# Autodesk Inventor assembly: SPE3V1 Freno
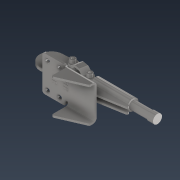
[picture p0: Inventor's stored thumbnail of the model, 180x180]
Saved by Autodesk Inventor 2021.2 (Build 252289000, 289)
## iProperties
Created: 2026-06-23
Part Number: SPE3V1 Freno
Document SubType Name: Assembly
Designer: nelso
Author: nelso
## Documents named in this file (9)
- C:\Users\Tecnica\OneDrive\Documentos\Mecanica\Soporte-Paciente-Espinografia\Workspace\SPE3V1 Freno.iam
- C:\Users\Tecnica\OneDrive\Documentos\Mecanica\Soporte-Paciente-Espinografia\Workspace\SP10V1 Estructura Freno.ipt
- C:\Users\Tecnica\OneDrive\Documentos\Mecanica\Soporte-Paciente-Espinografia\Workspace\SP9V1 Columna Freno.ipt
- C:\Users\Tecnica\OneDrive\Documentos\Mecanica\Soporte-Paciente-Espinografia\Workspace\SP5V1 Camisa Freno.ipt
- C:\Users\Tecnica\OneDrive\Documentos\Mecanica\Soporte-Paciente-Espinografia\Workspace\SP8V1 Conductor Hexagonal Freno.ipt
- C:\Users\Tecnica\OneDrive\Documentos\Mecanica\Soporte-Paciente-Espinografia\Workspace\SP6V1 Vastago Freno.ipt
- C:\Users\Tecnica\OneDrive\Documentos\Mecanica\Soporte-Paciente-Espinografia\Workspace\DIN912-M5X0.8L16P.ipt
- C:\Users\Tecnica\OneDrive\Documentos\Mecanica\Soporte-Paciente-Espinografia\Workspace\SP7V1 Viela Freno.ipt
- C:\Users\Tecnica\OneDrive\Documentos\Mecanica\Soporte-Paciente-Espinografia\Workspace\DIN555-5M5X0.8C.ipt
## Components (12 placed, 8 different names)
1. SP10V1 Estructura Freno:1 — Mate:5, Flush:2, Mate:11, Mate:13, Mate:35, Mate:46, Mate:58
2. SP9V1 Columna Freno:1 — Mate:13, Flush:3, Mate:46, Flush:5
3. SP9V1 Columna Freno:2 — Mate:11, Flush:4, Tangent:1, Mate:58
4. SP8V1 Conductor Hexagonal Freno:1 — Mate:34, Mate:38, Mate:62, Mate:71, Mate:74
5. SP6V1 Vastago Freno:1 — Mate:41, Mate:57, Flush:6, Mate:68
6. SP5V1 Camisa Freno:1 — Mate:33, Mate:40, Tangent:1, Flush:5, Mate:57, Flush:6
7. DIN912-M5X0.8L16P:1 — Mate:62, Mate:69, Mate:72, Mate:75, Mate:77
8. DIN912-M5X0.8L16P:2 — Mate:68, Mate:70, Mate:73, Mate:76, Mate:80
9. SP7V1 Viela Freno:1 — Mate:69, Mate:70, Mate:71, Mate:78, Mate:79
10. SP7V1 Viela Freno:2 — Mate:72, Mate:73, Mate:74, Mate:75, Mate:76
11. DIN555-5M5X0.8C:1 — Mate:77, Mate:78
12. DIN555-5M5X0.8C:2 — Mate:79, Mate:80
## Relationships (32: Mate 26, Flush 5, Tangent 1)
- Mate:5: SP10V1 Estructura Freno:1
- Flush:2: SP10V1 Estructura Freno:1
- Mate:11: SP10V1 Estructura Freno:1 ↔ SP9V1 Columna Freno:2
- Mate:13: SP10V1 Estructura Freno:1 ↔ SP9V1 Columna Freno:1
- Mate:33: SP5V1 Camisa Freno:1
- Mate:34: SP8V1 Conductor Hexagonal Freno:1
- Flush:3 (4 mm): SP9V1 Columna Freno:1
- Mate:35: SP10V1 Estructura Freno:1
- Flush:4 (-4 mm): SP9V1 Columna Freno:2
- Mate:38: SP8V1 Conductor Hexagonal Freno:1
- Mate:40: SP5V1 Camisa Freno:1
- Tangent:1: SP9V1 Columna Freno:2 ↔ SP5V1 Camisa Freno:1
- Mate:41: SP6V1 Vastago Freno:1
- Mate:46: SP10V1 Estructura Freno:1 ↔ SP9V1 Columna Freno:1
- Flush:5: SP9V1 Columna Freno:1 ↔ SP5V1 Camisa Freno:1
- Mate:57: SP6V1 Vastago Freno:1 ↔ SP5V1 Camisa Freno:1
- Flush:6 (-18 mm): SP6V1 Vastago Freno:1 ↔ SP5V1 Camisa Freno:1
- Mate:58: SP10V1 Estructura Freno:1 ↔ SP9V1 Columna Freno:2
- Mate:62: SP8V1 Conductor Hexagonal Freno:1 ↔ DIN912-M5X0.8L16P:1
- Mate:68: SP6V1 Vastago Freno:1 ↔ DIN912-M5X0.8L16P:2
- Mate:69: DIN912-M5X0.8L16P:1 ↔ SP7V1 Viela Freno:1
- Mate:70: DIN912-M5X0.8L16P:2 ↔ SP7V1 Viela Freno:1
- Mate:71: SP8V1 Conductor Hexagonal Freno:1 ↔ SP7V1 Viela Freno:1
- Mate:72: DIN912-M5X0.8L16P:1 ↔ SP7V1 Viela Freno:2
- Mate:73: DIN912-M5X0.8L16P:2 ↔ SP7V1 Viela Freno:2
- Mate:74: SP8V1 Conductor Hexagonal Freno:1 ↔ SP7V1 Viela Freno:2
- Mate:75: DIN912-M5X0.8L16P:1 ↔ SP7V1 Viela Freno:2
- Mate:76: DIN912-M5X0.8L16P:2 ↔ SP7V1 Viela Freno:2
- Mate:77: DIN912-M5X0.8L16P:1 ↔ DIN555-5M5X0.8C:1
- Mate:78: SP7V1 Viela Freno:1 ↔ DIN555-5M5X0.8C:1
- Mate:79: SP7V1 Viela Freno:1 ↔ DIN555-5M5X0.8C:2
- Mate:80: DIN912-M5X0.8L16P:2 ↔ DIN555-5M5X0.8C:2
